# Autodesk Inventor assembly: Assembly rc car
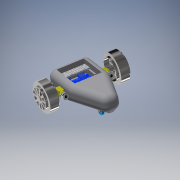
[picture p0: Inventor's stored thumbnail of the model, 180x180]
Saved by Autodesk Inventor 2019 (Build 230136000, 136)
## iProperties
Created: 2020-12-10
Part Number: Assembly rc car
Document SubType Name: Assembly
Designer: Victor Jiang
Author: Victor Jiang
## Documents named in this file (10)
- D:\Assembly rc car.iam
- D:\RC Car Chassis.ipt
- D:\Wheel for rc car.ipt
- D:\ardino.ipt
- D:\motor.ipt
- D:\straw.ipt
- D:\staw base.ipt
- D:\Wheel.ipt
- D:\straw v2.ipt
- D:\protoboard.ipt
## Components (12 placed, 9 different names)
1. RC Car Chassis:1 — Mate:1, Mate:2, Mate:3, Mate:4, Angle:1, Mate:7, Mate:8, Mate:16, Mate:19, Mate:20, Mate:22, Mate:23, Angle:2, Mate:24, Mate:25
2. Wheel for rc car:1 — Mate:14, Mate:15
3. Wheel for rc car:2 — Mate:12, Mate:13
4. ardino:1 — Mate:16, Mate:17, Mate:18
5. motor:1 — Mate:10, Mate:12, Mate:14, Mate:15, Mate:23
6. motor:2 — Mate:6, Angle:1, Mate:7, Mate:13
7. straw:1 — Mate:4, Mate:5, Mate:6
8. staw base:1 — Mate:1, Mate:2, Mate:3, Mate:5, Mate:9, Mate:17, Mate:18, Mate:26
9. straw:2 — Mate:8, Mate:9, Mate:10
10. Wheel:1 — Mate:21, Mate:22, Angle:2
11. straw v2:1 — Mate:19, Mate:20, Mate:21
12. protoboard:1 — Mate:24, Mate:25, Mate:26
## Relationships (27: Mate 25, Angle 2)
- Mate:1: RC Car Chassis:1 ↔ staw base:1
- Mate:2: RC Car Chassis:1 ↔ staw base:1
- Mate:3: RC Car Chassis:1 ↔ staw base:1
- Mate:4: RC Car Chassis:1 ↔ straw:1
- Mate:5: straw:1 ↔ staw base:1
- Mate:6: motor:2 ↔ straw:1
- Angle:1 (0 deg): RC Car Chassis:1 ↔ motor:2
- Mate:7: RC Car Chassis:1 ↔ motor:2
- Mate:8: RC Car Chassis:1 ↔ straw:2
- Mate:9: staw base:1 ↔ straw:2
- Mate:10: motor:1 ↔ straw:2
- Mate:12: Wheel for rc car:2 ↔ motor:1
- Mate:13: Wheel for rc car:2 ↔ motor:2
- Mate:14: Wheel for rc car:1 ↔ motor:1
- Mate:15: Wheel for rc car:1 ↔ motor:1
- Mate:16: RC Car Chassis:1 ↔ ardino:1
- Mate:17: ardino:1 ↔ staw base:1
- Mate:18: ardino:1 ↔ staw base:1
- Mate:19: RC Car Chassis:1 ↔ straw v2:1
- Mate:20: RC Car Chassis:1 ↔ straw v2:1
- Mate:21: Wheel:1 ↔ straw v2:1
- Mate:22: RC Car Chassis:1 ↔ Wheel:1
- Mate:23: RC Car Chassis:1 ↔ motor:1
- Angle:2 (0 deg): RC Car Chassis:1 ↔ Wheel:1
- Mate:24: RC Car Chassis:1 ↔ protoboard:1
- Mate:25: RC Car Chassis:1 ↔ protoboard:1
- Mate:26: staw base:1 ↔ protoboard:1
